# Autodesk Inventor assembly: Spider
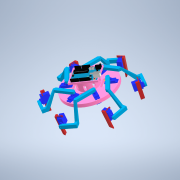
[picture p0: Inventor's stored thumbnail of the model, 180x180]
Saved by Autodesk Inventor 2022 (Build 260153000, 153)
## iProperties
Created: 2023-07-22
Part Number: Spider
Document SubType Name: Assembly
Designer: Eric Cao
Author: Eric Cao
## Documents named in this file (6)
- D:\CAD Practice\SpiderBot\Assemblies\Spider.iam
- D:\CAD Practice\SpiderBot\Drawings\Base.ipt
- D:\CAD Practice\SpiderBot\Drawings\Servo Motor.ipt
- D:\CAD Practice\SpiderBot\Drawings\leg.ipt
- D:\CAD Practice\SpiderBot\Drawings\connector.ipt
- D:\CAD Practice\SpiderBot\Parts\Arduino.ipt
## Components (26 placed, 5 different names)
1. Base:1 — Rigid:2, Rigid:3
2. Arduino:1 — Rigid:3
3. Servo Motor:11 — Rigid:2
4. Servo Motor:23
5. Servo Motor:24
6. Servo Motor:25
7. Servo Motor:26
8. Servo Motor:27 — Rotational:1
9. connector:11 — Rotational:1, Rotational:2
10. Servo Motor:10 — Rigid:1, Rotational:2
11. leg:1 — Rigid:1
12. connector:12
13. Servo Motor:28
14. leg:2
15. connector:13
16. Servo Motor:29
17. leg:3
18. connector:14
19. Servo Motor:30
20. leg:4
21. connector:15
22. Servo Motor:31
23. leg:5
24. connector:16
25. Servo Motor:32
26. leg:6
## Component patterns: (6 elements, first: Servo Motor:11), (6 elements, first: connector:11 + Servo Motor:10 + leg:1)
## Relationships (5: WeldJoint 3, RevoluteJoint 2)
- Rigid:1 [WeldJoint]: Servo Motor:10 ↔ leg:1
- Rigid:2 [WeldJoint]: Base:1 ↔ Servo Motor:11
- Rotational:1 [RevoluteJoint]: Servo Motor:27 ↔ connector:11
- Rotational:2 [RevoluteJoint]: connector:11 ↔ Servo Motor:10
- Rigid:3 [WeldJoint]: Base:1 ↔ Arduino:1
